# Autodesk Inventor assembly: CarBot
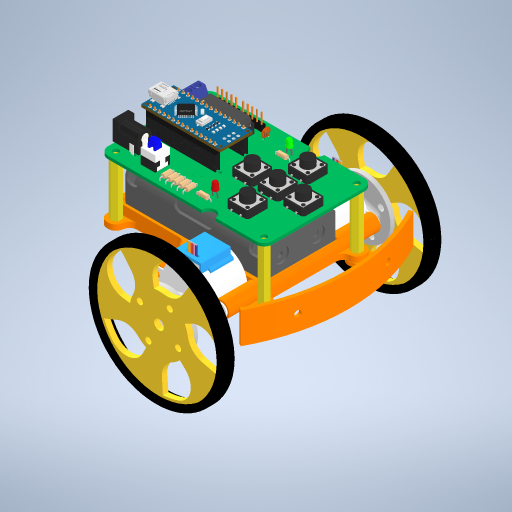
[picture p0: Inventor's stored thumbnail of the model, 512x512]
Saved by Autodesk Inventor 2023 (Build 270158000, 158)
## iProperties
Created: 2024-07-31
Part Number: CarBot
Document SubType Name: Assembly
Designer: LEGION
Author: LEGION
## Documents named in this file (11)
- E:\8 IDEX Pedro P. Diaz\4_Capacitaciones\2_Inventor\CarBot.iam
- E:\8 IDEX Pedro P. Diaz\4_Capacitaciones\1_Eagle\CarBot_3D\Componentes\28BYJ-48.ipt
- E:\8 IDEX Pedro P. Diaz\4_Capacitaciones\1_Eagle\CarBot_3D\Componentes\Bateria 2S.ipt
- E:\8 IDEX Pedro P. Diaz\4_Capacitaciones\1_Eagle\CarBot_3D\V2.0\CarBot_Pedro.iam
- E:\8 IDEX Pedro P. Diaz\4_Capacitaciones\2_Inventor\Llanta.ipt
- E:\8 IDEX Pedro P. Diaz\4_Capacitaciones\2_Inventor\Base.ipt
- E:\8 IDEX Pedro P. Diaz\4_Capacitaciones\2_Inventor\Varrilla_Cobre.ipt
- E:\8 IDEX Pedro P. Diaz\4_Capacitaciones\2_Inventor\Wheel_2D_Eje.ipt
- E:\8 IDEX Pedro P. Diaz\4_Capacitaciones\2_Inventor\Wheel_2D.iam
- E:\8 IDEX Pedro P. Diaz\4_Capacitaciones\2_Inventor\Decoracion\Soporte_Face.ipt
- E:\8 IDEX Pedro P. Diaz\4_Capacitaciones\2_Inventor\Decoracion\Face.ipt
## Components (17 placed, 10 different names)
1. 28BYJ-48:1 — Mate:4, Mate:5, Mate:6, Mate:26, Mate:27
2. 28BYJ-48:2 — Mate:1, Mate:2, Mate:3, Mate:25, Mate:28
3. Bateria 2S:1 — Mate:7, Mate:8
4. CarBot_Pedro:1 [sub-assembly] — Mate:18
5. Llanta:1 — Mate:15
6. Base:1 — Mate:1, Mate:2, Mate:3, Mate:4, Mate:5, Mate:6, Mate:7, Mate:8, Mate:15, Mate:16, Mate:17, Mate:19, Mate:20, Mate:21, Mate:22, Mate:23, Mate:24, Mate:35, Mate:36, Mate:37, Mate:38, Mate:39, Mate:40
7. Varrilla_Cobre:1 — Mate:16, Mate:17, Mate:18
8. Varrilla_Cobre:2 — Mate:23, Mate:24
9. Varrilla_Cobre:3 — Mate:19, Mate:20
10. Varrilla_Cobre:4 — Mate:21, Mate:22
11. Wheel_2D_Eje:1 — Mate:25, Mate:28, Mate:29, Mate:33, Mate:34
12. Wheel_2D_Eje:2 — Mate:26, Mate:27, Mate:30, Mate:31, Mate:32
13. Wheel_2D:1 [sub-assembly] — Mate:29, Mate:33, Mate:34
14. Wheel_2D:2 [sub-assembly] — Mate:30, Mate:31, Mate:32
15. Soporte_Face:1 — Mate:35, Mate:36, Mate:37, Mate:41, Flush:1
16. Soporte_Face:2 — Mate:38, Mate:39, Mate:40
17. Face:1 — Mate:41, Flush:1
## Relationships (36: Mate 35, Flush 1)
- Mate:1: 28BYJ-48:2 ↔ Base:1
- Mate:2: 28BYJ-48:2 ↔ Base:1
- Mate:3: 28BYJ-48:2 ↔ Base:1
- Mate:4: 28BYJ-48:1 ↔ Base:1
- Mate:5: 28BYJ-48:1 ↔ Base:1
- Mate:6: 28BYJ-48:1 ↔ Base:1
- Mate:7: Bateria 2S:1 ↔ Base:1
- Mate:8 (2.5 mm): Bateria 2S:1 ↔ Base:1
- Mate:15: Llanta:1 ↔ Base:1
- Mate:16: Base:1 ↔ Varrilla_Cobre:1
- Mate:17: Base:1 ↔ Varrilla_Cobre:1
- Mate:18: CarBot_Pedro:1 ↔ Varrilla_Cobre:1
- Mate:19: Base:1 ↔ Varrilla_Cobre:3
- Mate:20: Base:1 ↔ Varrilla_Cobre:3
- Mate:21: Base:1 ↔ Varrilla_Cobre:4
- Mate:22: Base:1 ↔ Varrilla_Cobre:4
- Mate:23: Base:1 ↔ Varrilla_Cobre:2
- Mate:24: Base:1 ↔ Varrilla_Cobre:2
- Mate:25: 28BYJ-48:2 ↔ Wheel_2D_Eje:1
- Mate:26: 28BYJ-48:1 ↔ Wheel_2D_Eje:2
- Mate:27: 28BYJ-48:1 ↔ Wheel_2D_Eje:2
- Mate:28: 28BYJ-48:2 ↔ Wheel_2D_Eje:1
- Mate:29: Wheel_2D_Eje:1 ↔ Wheel_2D:1
- Mate:30: Wheel_2D_Eje:2 ↔ Wheel_2D:2
- Mate:31: Wheel_2D_Eje:2 ↔ Wheel_2D:2
- Mate:32: Wheel_2D_Eje:2 ↔ Wheel_2D:2
- Mate:33: Wheel_2D_Eje:1 ↔ Wheel_2D:1
- Mate:34: Wheel_2D_Eje:1 ↔ Wheel_2D:1
- Mate:35: Base:1 ↔ Soporte_Face:1
- Mate:36: Base:1 ↔ Soporte_Face:1
- Mate:37: Base:1 ↔ Soporte_Face:1
- Mate:38: Base:1 ↔ Soporte_Face:2
- Mate:39: Base:1 ↔ Soporte_Face:2
- Mate:40: Base:1 ↔ Soporte_Face:2
- Mate:41: Soporte_Face:1 ↔ Face:1
- Flush:1: Soporte_Face:1 ↔ Face:1
